# Autodesk Inventor assembly: CilindroHidraulico
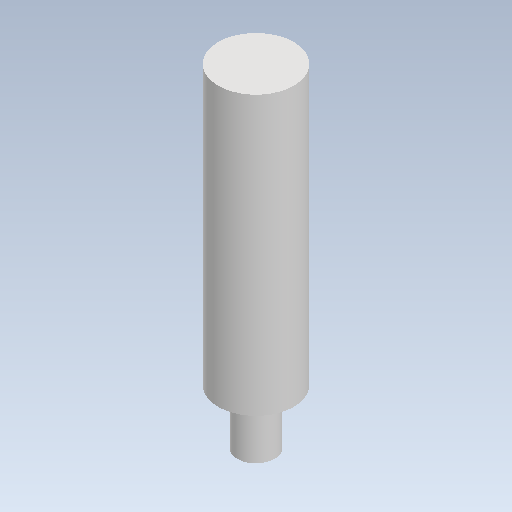
[picture p0: Inventor's stored thumbnail of the model, 512x512]
Saved by Autodesk Inventor 2021 (Build 250183000, 183)
## iProperties
Created: 2021-07-12
Part Number: CilindroHidraulico
Document SubType Name: Assembly
Designer: Nelson
Author: Nelson
## Documents named in this file (3)
- C:\Users\Nelson\Github\Proyecto_APM\CADs estaciones a automatizar\Estación mecanizado_boca de pescado\CilindroHidraulico.iam
- C:\Users\Nelson\Github\Proyecto_APM\CADs estaciones a automatizar\Estación mecanizado_boca de pescado\CilindroHidraulico_1.ipt
- C:\Users\Nelson\Github\Proyecto_APM\CADs estaciones a automatizar\Estación mecanizado_boca de pescado\CilindroHidraulico_2.ipt
## Components (2 placed, 2 different names)
1. CilindroHidraulico_1:1 — Mate:1, Flush:1
2. CilindroHidraulico_2:1 — Mate:1, Flush:1
## Relationships (2: Mate 1, Flush 1)
- Mate:1: CilindroHidraulico_1:1 ↔ CilindroHidraulico_2:1
- Flush:1 (130 mm): CilindroHidraulico_1:1 ↔ CilindroHidraulico_2:1
